# Autodesk Inventor assembly: fullbody
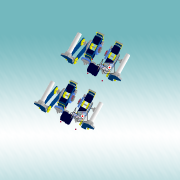
[picture p0: Inventor's stored thumbnail of the model, 180x180]
Saved by Autodesk Inventor 2020 (Build 240168000, 168)
## iProperties
Created: 2022-11-17
Part Number: fullbody
Document SubType Name: Assembly
Designer: kanazawakotaro
Author: kanazawakotaro
## Documents named in this file (3)
- C:\Users\金澤航太郎\Documents\Inventor\kamuy2\fullbody.iam
- C:\Users\金澤航太郎\Documents\Inventor\kamuy2\VER2.0_MIR_CPY.iam
- C:\Users\金澤航太郎\Documents\Inventor\kamuy2\VER2.0_MIR_CPY_MIR.iam
## Components (4 placed, 2 different names)
1. VER2.0_MIR_CPY:1 [sub-assembly] — フラッシュ:14, フラッシュ:15, メイト:1
2. VER2.0_MIR_CPY_MIR:1 [sub-assembly] — フラッシュ:14, フラッシュ:15, メイト:1, フラッシュ:18, フラッシュ:19
3. VER2.0_MIR_CPY:2 [sub-assembly]
4. VER2.0_MIR_CPY_MIR:2 [sub-assembly] — フラッシュ:18, フラッシュ:19
## Relationships (8: Flush 6, Mate 2)
- フラッシュ:14 [Flush]: VER2.0_MIR_CPY:1 ↔ VER2.0_MIR_CPY_MIR:1
- フラッシュ:15 [Flush]: VER2.0_MIR_CPY:1 ↔ VER2.0_MIR_CPY_MIR:1
- メイト:1 [Mate]: VER2.0_MIR_CPY:1 ↔ VER2.0_MIR_CPY_MIR:1
- [Flush]: VER2.0_MIR_CPY:2 ↔ VER2.0_MIR_CPY_MIR:2
- [Flush]: VER2.0_MIR_CPY:2 ↔ VER2.0_MIR_CPY_MIR:2
- [Mate]: VER2.0_MIR_CPY:2 ↔ VER2.0_MIR_CPY_MIR:2
- フラッシュ:18 [Flush]: VER2.0_MIR_CPY_MIR:1 ↔ VER2.0_MIR_CPY_MIR:2
- フラッシュ:19 [Flush]: VER2.0_MIR_CPY_MIR:1 ↔ VER2.0_MIR_CPY_MIR:2
## Named parameters: d20_d16 = 0 mm, d21_d18 = 0 mm, d22_d19 = 0 mm
